# Autodesk Inventor assembly: CHA_006_DrivePulleyAssembly_MIR_MIR
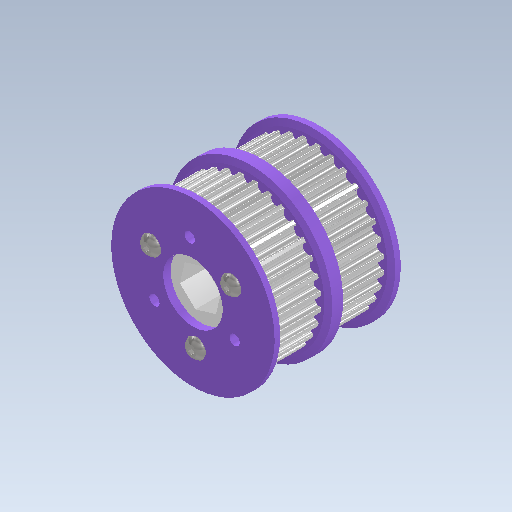
[picture p0: Inventor's stored thumbnail of the model, 512x512]
Saved by Autodesk Inventor 2020 (Build 240168000, 168)
## iProperties
Created: 2020-01-23
Part Number: CHA_006_DrivePulleyAssembly_MIR_MIR
Document SubType Name: Assembly
Designer: turnm
Mass: 80.3223 g
Surface Area: 341.903 cm^2
Volume: 73.8071 cm^3
Density: 1.08827 g/cm^3
Author: user
## Documents named in this file (5)
- C:\Users\turnm\Documents\GrabCAD\Infinite Recharge 2020\Build season\CHA_006_DrivePulleyAssembly_MIR_MIR.iam
- C:\Users\turnm\Documents\GrabCAD\Infinite Recharge 2020\Build season\CHA_003_DrivePulley_MIR_MIR.ipt
- C:\Users\turnm\Documents\GrabCAD\Infinite Recharge 2020\Build season\CHA_004_DrivePulleyFlange_MIR_MIR.ipt
- C:\Users\turnm\Documents\GrabCAD\Infinite Recharge 2020\Build season\CHA_005_DrivePulleyCenterFlange_MIR_MIR.ipt
- C:\Users\turnm\Documents\GrabCAD\Infinite Recharge 2020\Build season\CHA_008_PulleyScrew(6-32 0.5in)ButtonHeadScrew_MC-91255A148_MIR_MIR.ipt
## Components (11 placed, 4 different names)
1. CHA_003_DrivePulley_MIR_MIR:1 — Insert:1, Mate:2, Mate:3
2. CHA_003_DrivePulley_MIR_MIR:2 — Insert:2, Mate:1, Mate:8, Mate:7
3. CHA_004_DrivePulleyFlange_MIR_MIR:1 — Insert:2, Mate:1, Mate:6, Insert:7, Insert:6, Insert:8
4. CHA_004_DrivePulleyFlange_MIR_MIR:2 — Insert:1, Mate:2, Mate:6, Mate:8, Mate:4, Mate:5, Insert:3, Insert:4, Insert:5
5. CHA_005_DrivePulleyCenterFlange_MIR_MIR:1 — Mate:3, Mate:4, Mate:5, Mate:7
6. CHA_008_PulleyScrew(6-32 0.5in)ButtonHeadScrew_MC-91255A148_MIR_MIR:1 — Insert:3
7. CHA_008_PulleyScrew(6-32 0.5in)ButtonHeadScrew_MC-91255A148_MIR_MIR:2 — Insert:7
8. CHA_008_PulleyScrew(6-32 0.5in)ButtonHeadScrew_MC-91255A148_MIR_MIR:3 — Insert:6
9. CHA_008_PulleyScrew(6-32 0.5in)ButtonHeadScrew_MC-91255A148_MIR_MIR:4 — Insert:4
10. CHA_008_PulleyScrew(6-32 0.5in)ButtonHeadScrew_MC-91255A148_MIR_MIR:5 — Insert:8
11. CHA_008_PulleyScrew(6-32 0.5in)ButtonHeadScrew_MC-91255A148_MIR_MIR:6 — Insert:5
## Relationships (16: Insert 8, Mate 8)
- Insert:2: CHA_003_DrivePulley_MIR_MIR:2 ↔ CHA_004_DrivePulleyFlange_MIR_MIR:1
- Mate:1: CHA_003_DrivePulley_MIR_MIR:2 ↔ CHA_004_DrivePulleyFlange_MIR_MIR:1
- Insert:1: CHA_003_DrivePulley_MIR_MIR:1 ↔ CHA_004_DrivePulleyFlange_MIR_MIR:2
- Mate:2: CHA_003_DrivePulley_MIR_MIR:1 ↔ CHA_004_DrivePulleyFlange_MIR_MIR:2
- Mate:6: CHA_004_DrivePulleyFlange_MIR_MIR:1 ↔ CHA_004_DrivePulleyFlange_MIR_MIR:2
- Mate:8: CHA_003_DrivePulley_MIR_MIR:2 ↔ CHA_004_DrivePulleyFlange_MIR_MIR:2
- Mate:3: CHA_003_DrivePulley_MIR_MIR:1 ↔ CHA_005_DrivePulleyCenterFlange_MIR_MIR:1
- Mate:4: CHA_004_DrivePulleyFlange_MIR_MIR:2 ↔ CHA_005_DrivePulleyCenterFlange_MIR_MIR:1
- Mate:5: CHA_004_DrivePulleyFlange_MIR_MIR:2 ↔ CHA_005_DrivePulleyCenterFlange_MIR_MIR:1
- Mate:7: CHA_003_DrivePulley_MIR_MIR:2 ↔ CHA_005_DrivePulleyCenterFlange_MIR_MIR:1
- Insert:3: CHA_004_DrivePulleyFlange_MIR_MIR:2 ↔ CHA_008_PulleyScrew(6-32 0.5in)ButtonHeadScrew_MC-91255A148_MIR_MIR:1
- Insert:7: CHA_004_DrivePulleyFlange_MIR_MIR:1 ↔ CHA_008_PulleyScrew(6-32 0.5in)ButtonHeadScrew_MC-91255A148_MIR_MIR:2
- Insert:6: CHA_004_DrivePulleyFlange_MIR_MIR:1 ↔ CHA_008_PulleyScrew(6-32 0.5in)ButtonHeadScrew_MC-91255A148_MIR_MIR:3
- Insert:4: CHA_004_DrivePulleyFlange_MIR_MIR:2 ↔ CHA_008_PulleyScrew(6-32 0.5in)ButtonHeadScrew_MC-91255A148_MIR_MIR:4
- Insert:8: CHA_004_DrivePulleyFlange_MIR_MIR:1 ↔ CHA_008_PulleyScrew(6-32 0.5in)ButtonHeadScrew_MC-91255A148_MIR_MIR:5
- Insert:5: CHA_004_DrivePulleyFlange_MIR_MIR:2 ↔ CHA_008_PulleyScrew(6-32 0.5in)ButtonHeadScrew_MC-91255A148_MIR_MIR:6
